# Autodesk Inventor assembly: fab model mk-1
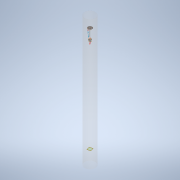
[picture p0: Inventor's stored thumbnail of the model, 180x180]
Saved by Autodesk Inventor 2020 (Build 240168000, 168)
## iProperties
Created: 2020-12-19
Part Number: fab model mk-1
Document SubType Name: Assembly
Designer: Vikki
Mass: 2463.35 g
Surface Area: 164488 cm^2
Volume: 40824.2 cm^3
Density: 0.0603404 g/cm^3
Author: Vikki
## Documents named in this file (27)
- E:\borewell rescuebot\pll manipulator files\sps manipulator\fab model mk-3 - new uv.iam
- E:\borewell rescuebot\pll manipulator files\sps manipulator\base.ipt
- E:\borewell rescuebot\pll manipulator files\sps manipulator\platform.ipt
- E:\borewell rescuebot\pll manipulator files\sps manipulator\leadscrew.ipt
- E:\borewell rescuebot\pll manipulator files\sps manipulator\coupler.ipt
- E:\borewell rescuebot\pll manipulator files\sps manipulator\telescopic boom1.ipt
- E:\borewell rescuebot\pll manipulator files\sps manipulator\boom 3.ipt
- E:\borewell rescuebot\pll manipulator files\sps manipulator\ball-pin.ipt
- E:\borewell rescuebot\2020 bot\borewell max sixe.ipt
- E:\borewell rescuebot\2020 bot\min size bore well.ipt
- E:\borewell rescuebot\pll manipulator files\sps manipulator\MicroGearmotor v3.ipt
- E:\borewell rescuebot\pll manipulator files\sps manipulator\plunger.ipt
- E:\borewell rescuebot\pll manipulator files\sps manipulator\piston.ipt
- E:\borewell rescuebot\pll manipulator files\sps manipulator\fab model mk-2\Design Accelerator\Bearing1.iam
- E:\borewell rescuebot\pll manipulator files\sps manipulator\fab model mk-2\Design Accelerator\Bearing2.iam
- E:\borewell rescuebot\pll manipulator files\sps manipulator\motor bracket n 20.ipt
- E:\borewell rescuebot\pll manipulator files\sps manipulator\female joint for uv.ipt
- E:\borewell rescuebot\pll manipulator files\sps manipulator\platform uv femal joint.ipt
- E:\borewell rescuebot\pll manipulator files\sps manipulator\boom to female.ipt
- E:\borewell rescuebot\pll manipulator files\sps manipulator\servo mg958 dummy.ipt
- E:\borewell rescuebot\pll manipulator files\sps manipulator\z roto base.ipt
- E:\borewell rescuebot\pll manipulator files\sps manipulator\MG-958 servo.iam
- E:\borewell rescuebot\pll manipulator files\sps manipulator\Tamiya SRB u joint.iam
- E:\borewell rescuebot\pll manipulator files\sps manipulator\fab model mk-3 - new uv\Design Accelerator\Bearing1.iam
- E:\borewell rescuebot\pll manipulator files\sps manipulator\loop catcher.ipt
- E:\borewell rescuebot\pll manipulator files\sps manipulator\base pin.ipt
- E:\borewell rescuebot\pll manipulator files\sps manipulator\platform pin for uv.ipt
## Components (43 placed, 24 different names)
1. base:1 — Mate:61, Flush:6, M1 C, Mate:161, Mate:162, Mate:163, Mate:164, Mate:165, Mate:166, Mate:167, Mate:168, Angle:16, Angle:17, Angle:18, Angle:19, $$a, Mate:187, Mate:188, Mate:189, Mate:190
2. platform:1 — M1 C, Mate:128, Mate:130, Angle:15, Mate:150, Flush:14, Mate:151, Mate:152, Flush:15, Flush:16, Mate:155, Mate:156, Angle:21, $$a, Angle:27, Mate:186, Mate:193, Mate:194
3. telescopic boom1:1 — Angle:12, Mate:140, Mate:149, Flush:17, Angle:20
4. boom 3:1 — Angle:12, Mate:149, Mate:173, Mate:174
5. ball-pin:1 — Mate:184, Mate:185
6. borewell max sixe:1 — Mate:61, Mate:62, Flush:5
7. min size bore well:1 — Mate:62, Flush:5, Flush:6
8. Bearing:4 [sub-assembly] — Mate:103, Flush:13, Mate:119
9. Bearing:5 [sub-assembly] — Mate:105, Flush:12
10. boom to female:1 — Mate:140, Flush:17, Mate:171, Mate:172
11. servo mg958 dummy:1
12. MicroGearmotor v3:2 — Mate:125, Mate:126, Angle:14
13. z roto base:1 — Mate:125, Mate:126, Angle:14, Mate:127, Mate:129, Mate:180, Mate:181, Angle:23, Angle:27
14. MG-958 servo:1 [sub-assembly] — Mate:127, Mate:128, Mate:129, Mate:130, Angle:15
15. Bearing:6 [sub-assembly] — Mate:150, Flush:14, Mate:157, Mate:158
16. Bearing:7 [sub-assembly] — Mate:152, Flush:15, Mate:153, Mate:154, Mate:191, Mate:192
17. Bearing:8 [sub-assembly] — Mate:151, Flush:16, Mate:159, Mate:160
18. Tamiya SRB u joint:1 [sub-assembly] — Mate:153, Mate:154, Mate:179
19. Tamiya SRB u joint:2 [sub-assembly] — Mate:155, Mate:156, Mate:173, Mate:174, Angle:21, Angle:22
20. Tamiya SRB u joint:3 [sub-assembly] — Mate:159, Mate:160, Mate:178
21. Tamiya SRB u joint:4 [sub-assembly] — Mate:157, Mate:158, Mate:175, Mate:176
22. Tamiya SRB u joint:5 [sub-assembly] — Mate:161, Mate:162, Angle:18, Mate:178
23. Tamiya SRB u joint:6 [sub-assembly] — Mate:165, Mate:166, Angle:16, Mate:169, Mate:170, Angle:24
24. Tamiya SRB u joint:7 [sub-assembly] — Mate:167, Mate:168, Angle:17, Mate:171, Mate:172, Angle:20, Angle:22
25. Tamiya SRB u joint:8 [sub-assembly] — Mate:163, Mate:164, Angle:19, Mate:179
26. loop catcher:1 — Mate:180, Mate:181, Angle:23, Mate:184, Mate:185
27. platform uv femal joint:1 — Mate:113, Mate:139, Mate:175, Mate:176
28. plunger:1 — Mate:97, Angle:11, Mate:113, Mate:139
29. female joint for uv:1 — Mate:110, Mate:138, Mate:169, Mate:170
30. MicroGearmotor v3:1 — Mate:95, Mate:98, Angle:9, Mate:120, Angle:25, Mate:183
31. leadscrew:1 — Mate:37, Mate:97, Mate:103, Angle:25, Angle:26, Mate:183
32. coupler:1 — Mate:37, Mate:95, Mate:105, Mate:118, Mate:119, Angle:26
33. piston:1 — Mate:98, Angle:10, Angle:11, Mate:117
34. motor bracket n 20:1 — Angle:9, Mate:110, Flush:12, Angle:10, Mate:117, Flush:13, Mate:118, Mate:120, Mate:138, Angle:24
35. ball-pin:2 — Mate:186
36. base pin:4 — Mate:189, Mate:190
37. platform pin for uv:4 — Mate:193, Mate:194
38. base pin:1 — Mate:187, Mate:188
39. base pin:2
40. base pin:3
41. platform pin for uv:1 — Mate:191, Mate:192
42. platform pin for uv:2
43. platform pin for uv:3
## Component patterns: (3 elements, first: base pin:1), (3 elements, first: platform pin for uv:1)
## Relationships (97: Mate 68, Angle 18, Flush 11)
- Mate:37: leadscrew:1 ↔ coupler:1
- [Flush]: borewell max sixe:1 ↔ min size bore well:1
- [Flush]: borewell max sixe:1 ↔ min size bore well:1
- Mate:61: base:1 ↔ borewell max sixe:1
- Mate:62: borewell max sixe:1 ↔ min size bore well:1
- Flush:5: borewell max sixe:1 ↔ min size bore well:1
- Flush:6 (-400 mm): base:1 ↔ min size bore well:1
- M1 C [Flush] (350 mm): base:1 ↔ platform:1
- Mate:95: MicroGearmotor v3:1 ↔ coupler:1
- Mate:97: plunger:1 ↔ leadscrew:1
- Mate:98: MicroGearmotor v3:1 ↔ piston:1
- Mate:103: Bearing:4 ↔ leadscrew:1
- Mate:105: Bearing:5 ↔ coupler:1
- Angle:9 (0 deg): MicroGearmotor v3:1 ↔ motor bracket n 20:1
- Mate:110: female joint for uv:1 ↔ motor bracket n 20:1
- Flush:12: Bearing:5 ↔ motor bracket n 20:1
- Angle:10 (0 deg): piston:1 ↔ motor bracket n 20:1
- Angle:11 (0 deg): plunger:1 ↔ piston:1
- Mate:113: platform uv femal joint:1 ↔ plunger:1
- Angle:12 (0 deg): telescopic boom1:1 ↔ boom 3:1
- Mate:117: piston:1 ↔ motor bracket n 20:1
- Flush:13: Bearing:4 ↔ motor bracket n 20:1
- Mate:118: coupler:1 ↔ motor bracket n 20:1
- Mate:119: Bearing:4 ↔ coupler:1
- Mate:120: MicroGearmotor v3:1 ↔ motor bracket n 20:1
- Mate:125: MicroGearmotor v3:2 ↔ z roto base:1
- Mate:126: MicroGearmotor v3:2 ↔ z roto base:1
- Angle:14 (180 deg): MicroGearmotor v3:2 ↔ z roto base:1
- Mate:127: z roto base:1 ↔ MG-958 servo:1
- Mate:128: platform:1 ↔ MG-958 servo:1
- Mate:129 (3 mm): z roto base:1 ↔ MG-958 servo:1
- Mate:130: platform:1 ↔ MG-958 servo:1
- Angle:15 (0 deg): platform:1 ↔ MG-958 servo:1
- Mate:138: female joint for uv:1 ↔ motor bracket n 20:1
- Mate:139: platform uv femal joint:1 ↔ plunger:1
- Mate:140: telescopic boom1:1 ↔ boom to female:1
- Mate:149: telescopic boom1:1 ↔ boom 3:1
- Mate:150: platform:1 ↔ Bearing:6
- Flush:14: platform:1 ↔ Bearing:6
- Mate:151: platform:1 ↔ Bearing:8
- Mate:152: platform:1 ↔ Bearing:7
- Flush:15: platform:1 ↔ Bearing:7
- Flush:16: platform:1 ↔ Bearing:8
- Flush:17: telescopic boom1:1 ↔ boom to female:1
- Mate:153: Bearing:7 ↔ Tamiya SRB u joint:1
- Mate:154: Bearing:7 ↔ Tamiya SRB u joint:1
- Mate:155: platform:1 ↔ Tamiya SRB u joint:2
- Mate:156: platform:1 ↔ Tamiya SRB u joint:2
- Mate:157: Bearing:6 ↔ Tamiya SRB u joint:4
- Mate:158: Bearing:6 ↔ Tamiya SRB u joint:4
- Mate:159: Bearing:8 ↔ Tamiya SRB u joint:3
- Mate:160: Bearing:8 ↔ Tamiya SRB u joint:3
- Mate:161: base:1 ↔ Tamiya SRB u joint:5
- Mate:162: base:1 ↔ Tamiya SRB u joint:5
- Mate:163: base:1 ↔ Tamiya SRB u joint:8
- Mate:164: base:1 ↔ Tamiya SRB u joint:8
- Mate:165: base:1 ↔ Tamiya SRB u joint:6
- Mate:166: base:1 ↔ Tamiya SRB u joint:6
- Mate:167: base:1 ↔ Tamiya SRB u joint:7
- Mate:168: base:1 ↔ Tamiya SRB u joint:7
- Angle:16 (30 deg): base:1 ↔ Tamiya SRB u joint:6
- Mate:169: Tamiya SRB u joint:6 ↔ female joint for uv:1
- Mate:170: Tamiya SRB u joint:6 ↔ female joint for uv:1
- Angle:17 (0 deg): base:1 ↔ Tamiya SRB u joint:7
- Angle:18 (0 deg): base:1 ↔ Tamiya SRB u joint:5
- Angle:19 (240 deg): base:1 ↔ Tamiya SRB u joint:8
- Mate:171: boom to female:1 ↔ Tamiya SRB u joint:7
- Mate:172: boom to female:1 ↔ Tamiya SRB u joint:7
- Angle:20 (0 deg): telescopic boom1:1 ↔ Tamiya SRB u joint:7
- Mate:173: boom 3:1 ↔ Tamiya SRB u joint:2
- Mate:174: boom 3:1 ↔ Tamiya SRB u joint:2
- Angle:21 (30 deg): platform:1 ↔ Tamiya SRB u joint:2
- Angle:22 (0 deg): Tamiya SRB u joint:2 ↔ Tamiya SRB u joint:7
- Mate:175: Tamiya SRB u joint:4 ↔ platform uv femal joint:1
- Mate:176: Tamiya SRB u joint:4 ↔ platform uv femal joint:1
- Mate:178: Tamiya SRB u joint:3 ↔ Tamiya SRB u joint:5
- Mate:179: Tamiya SRB u joint:1 ↔ Tamiya SRB u joint:8
- Mate:180: z roto base:1 ↔ loop catcher:1
- Mate:181: z roto base:1 ↔ loop catcher:1
- Angle:23 (0 deg): z roto base:1 ↔ loop catcher:1
- $$a [Mate]: base:1 ↔ platform:1
- Angle:24 (270 deg): Tamiya SRB u joint:6 ↔ motor bracket n 20:1
- Angle:25 (0 deg): MicroGearmotor v3:1 ↔ leadscrew:1
- Angle:26 (180 deg): leadscrew:1 ↔ coupler:1
- Mate:183: MicroGearmotor v3:1 ↔ leadscrew:1
- Angle:27 (0 deg): platform:1 ↔ z roto base:1
- Mate:184: ball-pin:1 ↔ loop catcher:1
- Mate:185: ball-pin:1 ↔ loop catcher:1
- Mate:186: platform:1 ↔ ball-pin:2
- Mate:187: base:1 ↔ base pin:1
- Mate:188: base:1 ↔ base pin:1
- Mate:189: base:1 ↔ base pin:4
- Mate:190: base:1 ↔ base pin:4
- Mate:191: Bearing:7 ↔ platform pin for uv:1
- Mate:192: Bearing:7 ↔ platform pin for uv:1
- Mate:193: platform:1 ↔ platform pin for uv:4
- Mate:194: platform:1 ↔ platform pin for uv:4
